# Autodesk Inventor assembly: ShinGuardTest
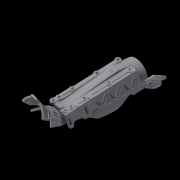
[picture p0: Inventor's stored thumbnail of the model, 180x180]
Saved by Autodesk Inventor 2015 (Build 190159000, 159)
## iProperties
Created: 2015-05-15
Part Number: ShinGuardTest
Document SubType Name: Assembly
Designer: Val
Author: Val
## Documents named in this file (8)
- F:\Exo\Models\3D\ShinRight.iam
- F:\Exo\Models\3D\Shin.ipt
- F:\Exo\Models\3D\ShinShockPlateRight.ipt
- F:\Exo\Models\3D\ShinLockRight.ipt
- F:\Exo\Models\3D\ShinConnectorLeft.ipt
- F:\Exo\Models\3D\ShinExtender.ipt
- F:\Exo\Models\3D\FootShockPlate.ipt
- F:\Exo\Models\3D\FootUpperShockPlate.ipt
## Components (7 placed, 7 different names)
1. ShinGuardRight:1 — Mate:1, Mate:2, Mate:3, Mate:4, Mate:5, Mate:6, Mate:9, Mate:10, Mate:11
2. ShinShockPlateRight:1 — Mate:1, Mate:2, Mate:3
3. ShinLockRight:1 — Mate:4, Mate:5, Mate:6
4. ShinConnectorLeft:1 — Mate:9, Mate:10, Mate:11, Mate:12, Mate:13, Mate:14
5. ShinExtender:1 — Mate:12, Mate:13, Mate:14
6. FootShockPlate:1
7. FootUpperShockPlate:1
## Relationships (12: Mate 12)
- Mate:1: ShinGuardRight:1 ↔ ShinShockPlateRight:1
- Mate:2: ShinGuardRight:1 ↔ ShinShockPlateRight:1
- Mate:3: ShinGuardRight:1 ↔ ShinShockPlateRight:1
- Mate:4: ShinGuardRight:1 ↔ ShinLockRight:1
- Mate:5: ShinGuardRight:1 ↔ ShinLockRight:1
- Mate:6: ShinGuardRight:1 ↔ ShinLockRight:1
- Mate:9: ShinGuardRight:1 ↔ ShinConnectorLeft:1
- Mate:10: ShinGuardRight:1 ↔ ShinConnectorLeft:1
- Mate:11: ShinGuardRight:1 ↔ ShinConnectorLeft:1
- Mate:12: ShinConnectorLeft:1 ↔ ShinExtender:1
- Mate:13: ShinConnectorLeft:1 ↔ ShinExtender:1
- Mate:14: ShinConnectorLeft:1 ↔ ShinExtender:1
